# Autodesk Inventor assembly: FrameAssembly
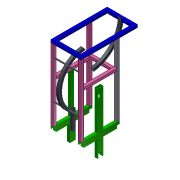
[picture p0: Inventor's stored thumbnail of the model, 180x180]
Saved by Autodesk Inventor 2012 (Build 160160000, 160)
## iProperties
Created: 2012-01-13
Part Number: FrameAssembly
Document SubType Name: Assembly
Designer: JesseK
Mass: 3933.14 g
Surface Area: 15477.6 cm^2
Volume: 1542.86 cm^3
Density: 2.54926 g/cm^3
Author: JesseK
## Documents named in this file (12)
- Z:\UserData\Documents\Inventor\team1885frc\Robot2012\Conveyor2\FrameAssembly.iam
- Z:\UserData\Documents\Inventor\team1885frc\Robot2012\Conveyor2\Frame_MainHorizontalMount.ipt
- Z:\UserData\Documents\Inventor\team1885frc\Robot2012\Conveyor2\Frame_LowerRollerMount.ipt
- Z:\UserData\Documents\Inventor\team1885frc\Robot2012\Conveyor2\Frame_UpperRollerMount.ipt
- Z:\UserData\Documents\Inventor\team1885frc\Robot2012\Conveyor2\Frame_MidRollerMount.ipt
- Z:\UserData\Documents\Inventor\team1885frc\Robot2012\Conveyor2\Frame_UpperFrameSupport.ipt
- Z:\UserData\Documents\Inventor\team1885frc\Robot2012\Conveyor2\Frame_UpperFrameSupport_Rear.ipt
- Z:\UserData\Documents\Inventor\team1885frc\Robot2012\Conveyor2\Shooter_Frame_FrontGuide.ipt
- Z:\UserData\Documents\Inventor\team1885frc\Robot2012\Conveyor2\Frame_UpperFrame.ipt
- Z:\UserData\Documents\Inventor\team1885frc\Robot2012\Conveyor2\Shooter_Frame_RearGuide.ipt
- Z:\UserData\Documents\Inventor\team1885frc\Robot2012\Conveyor2\Frame_UpperCrossFrame.ipt
- Z:\UserData\Documents\Inventor\team1885frc\Robot2012\Conveyor2\Frame_LowerConveyorBallSupport.ipt
## Components (19 placed, 11 different names)
1. Frame_MainHorizontalMount:1 — Mate:1, Flush:1, Flush:2, Mate:2, Mate:4, Flush:4, Mate:7, Flush:8, Mate:27, Mate:29, Flush:10, Flush:11, Mate:34
2. Frame_MainHorizontalMount:2 — Mate:1, Flush:1, Flush:2, Mate:6, Mate:16, Mate:17, Flush:6, Flush:7, Mate:26, Mate:28, Flush:12, Flush:13, Flush:29
3. Frame_LowerRollerMount:1 — Mate:2, Mate:4, Flush:4, Mate:8, Flush:5
4. Frame_UpperRollerMount:1 — Mate:6, Mate:7, Mate:8, Mate:43
5. Frame_MidRollerMount:1 — Mate:16, Mate:17, Flush:5
6. Frame_UpperFrameSupport:2 — Flush:6, Flush:7, Mate:26, Flush:9, Flush:19, Flush:20, Mate:36, Flush:26
7. Frame_UpperFrameSupport:4 — Flush:8, Flush:9, Mate:27, Flush:16, Mate:33, Flush:17, Flush:18, Mate:35
8. Frame_UpperFrameSupport:5 — Mate:29, Flush:10, Flush:11, Mate:30, Flush:14
9. Frame_UpperFrameSupport:6 — Mate:28, Flush:12, Flush:13, Mate:31, Flush:15, Mate:41, Flush:28
10. Frame_UpperFrameSupport_Rear:1 — Mate:31, Flush:15, Mate:44
11. Frame_UpperFrameSupport_Rear:2 — Mate:30, Flush:14, Mate:42, Mate:43
12. Shooter_Frame_FrontGuide:1 — Flush:16, Mate:33, Mate:34, Flush:21
13. Frame_UpperFrame:1 — Flush:17, Flush:18, Mate:35
14. Frame_UpperFrame:2 — Flush:19, Flush:20, Mate:36, Mate:38, Flush:23, Flush:24, Mate:39, Flush:25
15. Shooter_Frame_RearGuide:1 — Flush:21, Flush:27, Mate:40
16. Frame_UpperCrossFrame:1 — Mate:38, Flush:23, Flush:24, Flush:27, Mate:40
17. Frame_UpperCrossFrame:2 — Mate:39, Flush:25, Flush:26
18. Frame_UpperCrossFrame:3 — Mate:41, Flush:28, Mate:42, Mate:44
19. Frame_LowerConveyorBallSupport:1 — Flush:29
## Relationships (52: Flush 27, Mate 25)
- Mate:1 (228.6 mm): Frame_MainHorizontalMount:1 ↔ Frame_MainHorizontalMount:2
- Flush:1: Frame_MainHorizontalMount:1 ↔ Frame_MainHorizontalMount:2
- Flush:2: Frame_MainHorizontalMount:1 ↔ Frame_MainHorizontalMount:2
- Mate:2: Frame_MainHorizontalMount:1 ↔ Frame_LowerRollerMount:1
- Mate:4: Frame_MainHorizontalMount:1 ↔ Frame_LowerRollerMount:1
- Flush:4 (152.4 mm): Frame_MainHorizontalMount:1 ↔ Frame_LowerRollerMount:1
- Mate:6: Frame_MainHorizontalMount:2 ↔ Frame_UpperRollerMount:1
- Mate:7: Frame_MainHorizontalMount:1 ↔ Frame_UpperRollerMount:1
- Mate:8: Frame_LowerRollerMount:1 ↔ Frame_UpperRollerMount:1
- Mate:16: Frame_MainHorizontalMount:2 ↔ Frame_MidRollerMount:1
- Mate:17: Frame_MainHorizontalMount:2 ↔ Frame_MidRollerMount:1
- Flush:5: Frame_LowerRollerMount:1 ↔ Frame_MidRollerMount:1
- Flush:6: Frame_MainHorizontalMount:2 ↔ Frame_UpperFrameSupport:2
- Flush:7: Frame_MainHorizontalMount:2 ↔ Frame_UpperFrameSupport:2
- Mate:26: Frame_MainHorizontalMount:2 ↔ Frame_UpperFrameSupport:2
- Flush:8: Frame_MainHorizontalMount:1 ↔ Frame_UpperFrameSupport:4
- Flush:9: Frame_UpperFrameSupport:2 ↔ Frame_UpperFrameSupport:4
- Mate:27: Frame_MainHorizontalMount:1 ↔ Frame_UpperFrameSupport:4
- Mate:28: Frame_MainHorizontalMount:2 ↔ Frame_UpperFrameSupport:6
- Mate:29: Frame_MainHorizontalMount:1 ↔ Frame_UpperFrameSupport:5
- Flush:10: Frame_MainHorizontalMount:1 ↔ Frame_UpperFrameSupport:5
- Flush:11: Frame_MainHorizontalMount:1 ↔ Frame_UpperFrameSupport:5
- Flush:12: Frame_MainHorizontalMount:2 ↔ Frame_UpperFrameSupport:6
- Flush:13: Frame_MainHorizontalMount:2 ↔ Frame_UpperFrameSupport:6
- Mate:30: Frame_UpperFrameSupport:5 ↔ Frame_UpperFrameSupport_Rear:2
- Flush:14: Frame_UpperFrameSupport:5 ↔ Frame_UpperFrameSupport_Rear:2
- Mate:31: Frame_UpperFrameSupport:6 ↔ Frame_UpperFrameSupport_Rear:1
- Flush:15: Frame_UpperFrameSupport:6 ↔ Frame_UpperFrameSupport_Rear:1
- Flush:16 (127 mm): Frame_UpperFrameSupport:4 ↔ Shooter_Frame_FrontGuide:1
- Mate:33 (25.4 mm): Frame_UpperFrameSupport:4 ↔ Shooter_Frame_FrontGuide:1
- Mate:34: Frame_MainHorizontalMount:1 ↔ Shooter_Frame_FrontGuide:1
- Flush:17: Frame_UpperFrameSupport:4 ↔ Frame_UpperFrame:1
- Flush:18: Frame_UpperFrameSupport:4 ↔ Frame_UpperFrame:1
- Mate:35: Frame_UpperFrameSupport:4 ↔ Frame_UpperFrame:1
- Flush:19: Frame_UpperFrameSupport:2 ↔ Frame_UpperFrame:2
- Flush:20: Frame_UpperFrameSupport:2 ↔ Frame_UpperFrame:2
- Mate:36: Frame_UpperFrameSupport:2 ↔ Frame_UpperFrame:2
- Flush:21: Shooter_Frame_FrontGuide:1 ↔ Shooter_Frame_RearGuide:1
- Mate:38: Frame_UpperFrame:2 ↔ Frame_UpperCrossFrame:1
- Flush:23: Frame_UpperFrame:2 ↔ Frame_UpperCrossFrame:1
- Flush:24: Frame_UpperFrame:2 ↔ Frame_UpperCrossFrame:1
- Mate:39: Frame_UpperFrame:2 ↔ Frame_UpperCrossFrame:2
- Flush:25: Frame_UpperFrame:2 ↔ Frame_UpperCrossFrame:2
- Flush:26: Frame_UpperFrameSupport:2 ↔ Frame_UpperCrossFrame:2
- Flush:27: Shooter_Frame_RearGuide:1 ↔ Frame_UpperCrossFrame:1
- Mate:40: Shooter_Frame_RearGuide:1 ↔ Frame_UpperCrossFrame:1
- Mate:41: Frame_UpperFrameSupport:6 ↔ Frame_UpperCrossFrame:3
- Flush:28: Frame_UpperFrameSupport:6 ↔ Frame_UpperCrossFrame:3
- Flush:29: Frame_MainHorizontalMount:2 ↔ Frame_LowerConveyorBallSupport:1
- Mate:42: Frame_UpperFrameSupport_Rear:2 ↔ Frame_UpperCrossFrame:3
- Mate:43 (50.8 mm): Frame_UpperRollerMount:1 ↔ Frame_UpperFrameSupport_Rear:2
- Mate:44 (-12.7 mm): Frame_UpperFrameSupport_Rear:1 ↔ Frame_UpperCrossFrame:3
